# Autodesk Inventor assembly: atividade_14A_montagem
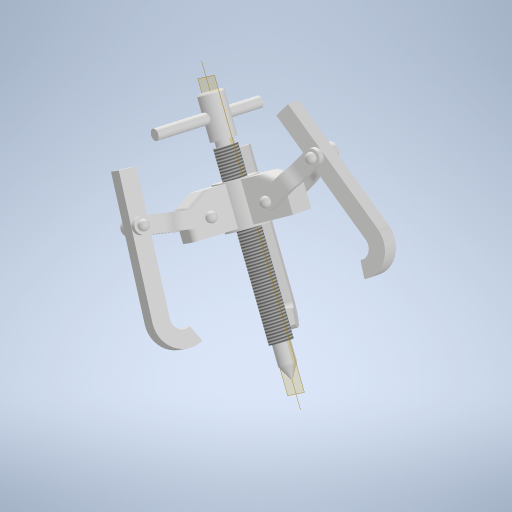
[picture p0: Inventor's stored thumbnail of the model, 512x512]
Saved by Autodesk Inventor 2024.2 (Build 282272000, 272)
## iProperties
Created: 2024-03-04
Part Number: atividade_14A_montagem
Document SubType Name: Assembly
Designer: 082220042
Author: 082220042
## Documents named in this file (8)
- Z:\EC_Engenharia_da_computacao\desenho_digital\atividade\atividade_14A\atividade_14A_montagem.iam
- Z:\EC_Engenharia_da_computacao\desenho_digital\atividade\atividade_14A\atividade_14A.ipt
- Z:\EC_Engenharia_da_computacao\desenho_digital\atividade\atividade_14A\atividade_14A_eixo.ipt
- Z:\EC_Engenharia_da_computacao\desenho_digital\atividade\atividade_14A\atividade_14A_garra.ipt
- Z:\EC_Engenharia_da_computacao\desenho_digital\atividade\atividade_14A\atividade_14A_pino_superior.ipt
- Z:\EC_Engenharia_da_computacao\desenho_digital\atividade\atividade_14A\atividade_14A_pino27.ipt
- Z:\EC_Engenharia_da_computacao\desenho_digital\atividade\atividade_14A\atividade_14A_pino37.ipt
- Z:\EC_Engenharia_da_computacao\desenho_digital\atividade\atividade_14A\atividade_14A_uniao.ipt
## Components (18 placed, 7 different names)
1. atividade_14A:1 — Cylindrical:1, Mate:1, Mate:2, Mate:3, Mate:8, Mate:9, Mate:11, Mate:12, Mate:13, Mate:14, Mate:15
2. atividade_14A_eixo:1 — Cylindrical:1, Mate:34
3. atividade_14A_garra:1 — Mate:20, Mate:21
4. atividade_14A_pino_superior:1 — Mate:34
5. atividade_14A_pino27:1 — Mate:26, Mate:27
6. atividade_14A_pino37:1 — Mate:30, Mate:31
7. atividade_14A_uniao:1 — Mate:12, Mate:13, Mate:21, Mate:22, Mate:23
8. atividade_14A_garra:2 — Mate:4, Mate:5, Mate:6, Mate:7
9. atividade_14A_garra:3 — Mate:16, Mate:17, Mate:18, Mate:19
10. atividade_14A_pino27:2 — Mate:24, Mate:25
11. atividade_14A_pino27:3 — Mate:22, Mate:23
12. atividade_14A_pino37:2 — Mate:32, Mate:33
13. atividade_14A_pino37:3 — Mate:28, Mate:29
14. atividade_14A_uniao:2 — Mate:1, Mate:5, Mate:6, Mate:32, Mate:33
15. atividade_14A_uniao:3 — Mate:11, Mate:18, Mate:19
16. atividade_14A_uniao:4 — Mate:8, Mate:9, Mate:16, Mate:17, Mate:26, Mate:27, Mate:28, Mate:29
17. atividade_14A_uniao:5 — Mate:2, Mate:3, Mate:4, Mate:7, Mate:24, Mate:25
18. atividade_14A_uniao:6 — Mate:14, Mate:15, Mate:20, Mate:30, Mate:31
## Relationships (34: Mate 33, CylindricalJoint 1)
- Cylindrical:1: atividade_14A:1 ↔ atividade_14A_eixo:1
- Mate:1: atividade_14A:1 ↔ atividade_14A_uniao:2
- Mate:2: atividade_14A:1 ↔ atividade_14A_uniao:5
- Mate:3: atividade_14A:1 ↔ atividade_14A_uniao:5
- Mate:4: atividade_14A_garra:2 ↔ atividade_14A_uniao:5
- Mate:5: atividade_14A_garra:2 ↔ atividade_14A_uniao:2
- Mate:6: atividade_14A_garra:2 ↔ atividade_14A_uniao:2
- Mate:7: atividade_14A_garra:2 ↔ atividade_14A_uniao:5
- Mate:8: atividade_14A:1 ↔ atividade_14A_uniao:4
- Mate:9: atividade_14A:1 ↔ atividade_14A_uniao:4
- Mate:11: atividade_14A:1 ↔ atividade_14A_uniao:3
- Mate:12: atividade_14A:1 ↔ atividade_14A_uniao:1
- Mate:13: atividade_14A:1 ↔ atividade_14A_uniao:1
- Mate:14: atividade_14A:1 ↔ atividade_14A_uniao:6
- Mate:15: atividade_14A:1 ↔ atividade_14A_uniao:6
- Mate:16: atividade_14A_garra:3 ↔ atividade_14A_uniao:4
- Mate:17: atividade_14A_garra:3 ↔ atividade_14A_uniao:4
- Mate:18: atividade_14A_garra:3 ↔ atividade_14A_uniao:3
- Mate:19: atividade_14A_garra:3 ↔ atividade_14A_uniao:3
- Mate:20: atividade_14A_garra:1 ↔ atividade_14A_uniao:6
- Mate:21: atividade_14A_garra:1 ↔ atividade_14A_uniao:1
- Mate:22: atividade_14A_uniao:1 ↔ atividade_14A_pino27:3
- Mate:23: atividade_14A_uniao:1 ↔ atividade_14A_pino27:3
- Mate:24: atividade_14A_pino27:2 ↔ atividade_14A_uniao:5
- Mate:25: atividade_14A_pino27:2 ↔ atividade_14A_uniao:5
- Mate:26: atividade_14A_pino27:1 ↔ atividade_14A_uniao:4
- Mate:27: atividade_14A_pino27:1 ↔ atividade_14A_uniao:4
- Mate:28: atividade_14A_pino37:3 ↔ atividade_14A_uniao:4
- Mate:29: atividade_14A_pino37:3 ↔ atividade_14A_uniao:4
- Mate:30: atividade_14A_pino37:1 ↔ atividade_14A_uniao:6
- Mate:31: atividade_14A_pino37:1 ↔ atividade_14A_uniao:6
- Mate:32: atividade_14A_pino37:2 ↔ atividade_14A_uniao:2
- Mate:33: atividade_14A_pino37:2 ↔ atividade_14A_uniao:2
- Mate:34: atividade_14A_eixo:1 ↔ atividade_14A_pino_superior:1
